# Autodesk Inventor assembly: Assembly
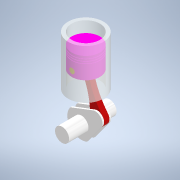
[picture p0: Inventor's stored thumbnail of the model, 180x180]
Saved by Autodesk Inventor 2021 (Build 250183000, 183)
## iProperties
Created: 2021-04-09
Part Number: Assembly
Document SubType Name: Assembly
Designer: tommy
Author: tommy
## Documents named in this file (5)
- C:\Users\tommy\Google Drive\ASME\CAD Workshop Spring 2021\Workshop Run 2\Assembly.iam
- C:\Users\tommy\Google Drive\ASME\CAD Workshop Spring 2021\Workshop Run 2\Sleeve.ipt
- C:\Users\tommy\Google Drive\ASME\CAD Workshop Spring 2021\Workshop Run 2\Piston.ipt
- C:\Users\tommy\Google Drive\ASME\CAD Workshop Spring 2021\Workshop Run 2\Crank_Shaft.ipt
- C:\Users\tommy\Google Drive\ASME\CAD Workshop Spring 2021\Workshop Run 2\Connecting_Rod.ipt
## Components (4 placed, 4 different names)
1. Sleeve:1 — Mate:4, Mate:5, Mate:6, Mate:7
2. Piston:1 — Mate:3, Flush:3, Mate:6
3. Crank_Shaft:1 — Mate:1, Flush:1, Mate:2, Angle:1
4. Connecting_Rod:1 — Mate:2, Flush:2, Mate:3
## Relationships (11: Mate 7, Flush 3, Angle 1)
- Mate:1: Crank_Shaft:1
- Flush:1: Crank_Shaft:1
- Mate:2: Crank_Shaft:1 ↔ Connecting_Rod:1
- Flush:2: Connecting_Rod:1
- Mate:3: Piston:1 ↔ Connecting_Rod:1
- Flush:3: Piston:1
- Mate:4: Sleeve:1
- Mate:5: Sleeve:1
- Mate:6: Sleeve:1 ↔ Piston:1
- Mate:7 (101.6 mm): Sleeve:1
- Angle:1 (0 deg): Crank_Shaft:1
